(part 1 of 2)
# Autodesk Inventor assembly: printer
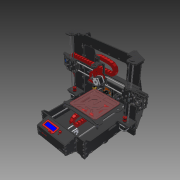
[picture p0: Inventor's stored thumbnail of the model, 180x180]
Saved by Autodesk Inventor 2014 (Build 180170000, 170)
## iProperties
Created: 2014-01-09
Part Number: printer
Document SubType Name: Assembly
Designer: buben
Author: buben
## Documents named in this file (53)
- C:\Users\buben\Documents\GitHub\bacon\inventor files\assemblies\printer.iam
- C:\Users\buben\Documents\GitHub\bacon\inventor files\printer parts\brace_left.ipt
- C:\Users\buben\Documents\GitHub\bacon\inventor files\printer parts\bottom.ipt
- C:\Users\buben\Documents\GitHub\bacon\inventor files\printer parts\brace_right.ipt
- C:\Users\buben\Documents\GitHub\bacon\inventor files\printer parts\front.ipt
- C:\Users\buben\Documents\GitHub\bacon\inventor files\printer parts\back.ipt
- C:\Users\buben\Documents\GitHub\bacon\inventor files\printer parts\frame.ipt
- C:\Users\buben\Documents\GitHub\bacon\inventor files\printer parts\z_motor_brace.ipt
- C:\Users\buben\Documents\GitHub\bacon\inventor files\printer parts\z_motor_mount.ipt
- C:\Users\buben\Documents\GitHub\bacon\inventor files\printer parts\y_axis_cap.ipt
- C:\Users\buben\Documents\GitHub\bacon\inventor files\printer parts\z_rod_stopper_bottom.ipt
- C:\Users\buben\Documents\GitHub\bacon\inventor files\3rd party components\nema_17_stepper\Imported Components\NEMA 17\NEMA 17.iam
- C:\Users\buben\Documents\GitHub\bacon\inventor files\utils\z_axis_rod.ipt
- C:\Users\buben\Documents\GitHub\bacon\inventor files\utils\z_threaded_rod.ipt
- C:\Users\buben\Documents\GitHub\bacon\inventor files\utils\y_axis_rod.ipt
- C:\Users\buben\Documents\GitHub\bacon\inventor files\printer parts\z_axis_top.ipt
- C:\Users\buben\Documents\GitHub\bacon\inventor files\printer parts\z_axis_top_cap.ipt
- C:\Users\buben\Documents\GitHub\bacon\inventor files\printer parts\frame_brace_top.ipt
- C:\Users\buben\Documents\GitHub\bacon\inventor files\utils\washer_m4.ipt
- C:\Users\buben\Documents\Inventor\Content Center Files\R2014\en-US\ISO 4762(2)\ISO 4762 - M4 x 20ISO.ipt
- C:\Users\buben\Documents\Inventor\Content Center Files\R2014\en-US\DIN 985\DIN 985 - M4.ipt
- C:\Users\buben\Documents\Inventor\Content Center Files\R2014\en-US\ISO 7040\ISO 7040 - M4.ipt
- C:\Users\buben\Documents\GitHub\bacon\inventor files\printer parts\wiring_brace.ipt
- C:\Users\buben\Documents\GitHub\bacon\inventor files\utils\washer_m3.ipt
- C:\Users\buben\Documents\Inventor\Content Center Files\R2014\en-US\ISO 4762(2)\ISO 4762 - M3 x 16ISO.ipt
- C:\Users\buben\Documents\GitHub\bacon\inventor files\3rd party components\PC Fan\Imported Components\PC Fan\PC Fan.iam
- C:\Users\buben\Documents\GitHub\bacon\inventor files\3rd party components\fan guard\Imported Components\User Library-Fan Guard\User Library-Fan Guard.ipt
- C:\Users\buben\Documents\GitHub\bacon\inventor files\printer parts\y_carriage_belt_iddler.ipt
- C:\Users\buben\Documents\GitHub\bacon\inventor files\printer parts\y_carriage_belt_iddler_holder.ipt
- C:\Users\buben\Documents\GitHub\bacon\inventor files\3rd party components\bearing_608\Imported Components\608RS\608RS.ipt
- C:\Users\buben\Documents\GitHub\bacon\inventor files\utils\belt_guide.ipt
- C:\Users\buben\Documents\GitHub\bacon\inventor files\utils\washer_m8.ipt
- C:\Users\buben\Documents\Inventor\Content Center Files\R2014\en-US\ISO 7040\ISO 7040 - M8.ipt
- C:\Users\buben\Documents\Inventor\Content Center Files\R2014\en-US\ISO 4762(2)\ISO 4762 - M8 x 40ISO.ipt
- C:\Users\buben\Documents\Inventor\Content Center Files\R2014\en-US\ISO 4762(2)\ISO 4762 - M4 x 30ISO.ipt
- C:\Users\buben\Documents\GitHub\bacon\inventor files\printer parts\y_motor_mount.ipt
- C:\Users\buben\Documents\GitHub\bacon\inventor files\printer parts\y_motor_mount_brace.ipt
- C:\Users\buben\Documents\GitHub\bacon\inventor files\printer parts\motor_spacer.ipt
- C:\Users\buben\Documents\GitHub\bacon\inventor files\3rd party components\nema_17_stepper\Imported Components\NEMA 17 with T5 Pulley\NEMA 17 with T5 Pulley.iam
- C:\Users\buben\Documents\GitHub\bacon\inventor files\assemblies\y_carryage.iam
- C:\Users\buben\Documents\GitHub\bacon\inventor files\assemblies\x_axis.iam
- C:\Users\buben\Documents\GitHub\bacon\inventor files\3rd party components\iec_plug_socket\Imported Components\IEC inlet\IEC inlet.ipt
- C:\Users\buben\Documents\GitHub\bacon\inventor files\utils\z_axis_cable_mount_b.ipt
- C:\Users\buben\Documents\GitHub\bacon\inventor files\utils\cable_chain_22.ipt
- C:\Users\buben\Documents\GitHub\bacon\inventor files\utils\z_axis_cable_mount_a.ipt
- C:\Users\buben\Documents\GitHub\bacon\inventor files\utils\y_axis_cable_mount_b.ipt
- C:\Users\buben\Documents\GitHub\bacon\inventor files\utils\x_axis_cable_mount_a.ipt
- C:\Users\buben\Documents\GitHub\bacon\inventor files\utils\z_axis_coupling_silicone_hose.ipt
- C:\Users\buben\Documents\GitHub\bacon\inventor files\printer parts\y_axis_cap_front_panel.ipt
- C:\Users\buben\Documents\GitHub\bacon\inventor files\assemblies\front_panel_2004.iam
- C:\Users\buben\Documents\GitHub\bacon\inventor files\utils\coupling_tie.ipt
- C:\Users\buben\Documents\GitHub\bacon\inventor files\utils\coupling_tie_belt.ipt
- C:\Users\buben\Documents\Inventor\Content Center Files\R2014\en-US\Screw F-Z GOST R ISO 7050-93\Screw ST4.2x16-F-Z GOST R ISO 7050-93.ipt
## Components (484 placed, 52 different names)
1. brace_left:1 — Mate:1, Mate:2, Mate:3, Mate:4, Mate:5, Flush:1, Mate:8, Mate:9, Mate:10, Mate:11, Mate:13, Mate:14, Mate:15, Mate:16, Mate:23, Mate:24, Mate:25, Mate:78, Mate:79, Flush:3, Mate:123, Mate:205, Mate:207, Mate:506, Flush:10
2. bottom:1 — Mate:4, Mate:5, Flush:1, Mate:6, Flush:2, Mate:7, Mate:12, Mate:80, Mate:91, Mate:484, Mate:485, Mate:510
3. brace_right:1 — Mate:6, Flush:2, Mate:7, Mate:26, Mate:28, Mate:70, Mate:90, Mate:184, Mate:202, Mate:204, Mate:211, Mate:212, Mate:341, Mate:342, Mate:360, Mate:500, Mate:501, Mate:502
4. front:1 — Mate:8, Mate:9, Mate:10, Mate:84, Mate:85, Mate:86, Mate:87, Mate:135, Mate:304, Mate:305, Mate:306, Mate:307, Mate:308, Mate:309, Mate:310, Mate:517, Mate:518, Mate:519, Mate:520, Angle:97, Angle:98, Mate:521, Mate:522, Mate:523, Mate:524, Mate:525, Mate:526, Mate:527, Mate:528, Mate:529, Mate:531, Mate:533, Mate:535, Mate:545, Flush:14, Mate:546
5. back:1 — Mate:11, Mate:12, Mate:13, Mate:35, Mate:36, Mate:37, Mate:38, Mate:39, Mate:40, Insert:3, Insert:4, Mate:255, Mate:256, Mate:257, Mate:258, Mate:286, Mate:287, Mate:288, Mate:289, Mate:290, Mate:291, Mate:292, Mate:511, Insert:188, Insert:189, Insert:190, Insert:191
6. frame:1 — Mate:14, Mate:15, Mate:16, Mate:17, Mate:18, Mate:19, Mate:20, Mate:21, Mate:22, Mate:27, Mate:57, Mate:58, Mate:59, Mate:60, Mate:61, Mate:62, Mate:69, Mate:71, Flush:4, Mate:121, Mate:122, Mate:168, Mate:169, Mate:170, Mate:171, Mate:172, Mate:173, Mate:203, Mate:206, Mate:208, Mate:209, Mate:362, Mate:364, Angle:99, Angle:100
7. z_motor_brace:1 — Mate:20, Mate:21, Mate:22
8. z_motor_brace:2 — Mate:17, Mate:18, Mate:19, Mate:174, Mate:176
9. z_motor_mount:1 — Mate:23, Mate:24, Mate:25, Mate:44, Mate:45, Mate:46, Mate:52, Insert:2
10. z_motor_mount:2 — Mate:26, Mate:27, Mate:28, Mate:41, Mate:42, Mate:43, Insert:1, Mate:160, Mate:161, Mate:162, Mate:163, Mate:164, Mate:165, Mate:166, Mate:167, Mate:180, Mate:182, Mate:220, Mate:221, Mate:222, Mate:223, Mate:224, Mate:225, Mate:226, Mate:227
11. y_axis_cap:2 — Mate:35, Mate:39, Mate:40
12. y_axis_cap:3 — Mate:36, Mate:37, Mate:38
13. z_rod_stopper_bottom:1 — Mate:44, Mate:45, Mate:46, Mate:50, Mate:51
14. z_rod_stopper_bottom:2 — Mate:41, Mate:42, Mate:43, Mate:47, Mate:48, Mate:49, Mate:178, Mate:186
15. NEMA 17:1 [sub-assembly] — Mate:47, Mate:48, Mate:49, Mate:53, Mate:54, Mate:514
16. NEMA 17:2 [sub-assembly] — Mate:50, Mate:51, Mate:52, Mate:55, Mate:56
17. z_axis_rod:1 — Insert:1, Mate:340
18. z_axis_rod:2 — Insert:2, Mate:339
19. z_threaded_rod:1 — Mate:55, Mate:56, Mate:515, Mate:516
20. z_threaded_rod:2 — Mate:53, Mate:54, Mate:513
21. y_axis_rod:1 — Insert:3, Mate:338
22. y_axis_rod:2 — Insert:4, Mate:337
23. z_axis_top:1 — Mate:57, Mate:58, Mate:59, Mate:63, Mate:67, Mate:68
24. z_axis_top:2 — Mate:60, Mate:61, Mate:62, Mate:64, Mate:65, Mate:66, Mate:354, Mate:355, Mate:356, Mate:357, Mate:358, Mate:359, Mate:366, Mate:368
25. z_axis_top_cap:1 — Mate:63, Mate:67, Mate:68
26. z_axis_top_cap:2 — Mate:64, Mate:65, Mate:66, Mate:350, Mate:351, Mate:352, Mate:353
27. frame_brace_top:1 — Mate:69, Mate:70, Mate:71, Mate:343
28. DIN 985 - replaced by DIN EN ISO 10511 M4:12
29. CSN 02 1702 B B 4,3:30 — Insert:9
30. CSN 02 1702 B B 4,3:31 — Mate:106, Mate:108
31. ISO 4762 M4 x 20:15 — Mate:106, Insert:9, Mate:107
32. DIN EN ISO 7040 M4:6 — Mate:107, Mate:108
33. DIN EN ISO 7040 M4:7
34. CSN 02 1702 B B 4,3:32
35. ISO 4762 M4 x 20:16
36. CSN 02 1702 B B 4,3:33
37. DIN EN ISO 7040 M4:8
38. CSN 02 1702 B B 4,3:34
39. ISO 4762 M4 x 20:17
40. CSN 02 1702 B B 4,3:35
41. CSN 02 1702 B B 4,3:42 — Insert:10
42. CSN 02 1702 B B 4,3:43 — Insert:11
43. CSN 02 1702 B B 4,3:44 — Mate:109, Mate:112
44. CSN 02 1702 B B 4,3:45 — Mate:110, Mate:114
45. ISO 4762 M4 x 20:21 — Mate:109, Insert:10, Mate:111
46. ISO 4762 M4 x 20:22 — Mate:110, Insert:11, Mate:113
47. DIN EN ISO 7040 M4:12 — Mate:111, Mate:112
48. DIN EN ISO 7040 M4:13 — Mate:113, Mate:114
49. DIN EN ISO 7040 M4:14
50. CSN 02 1702 B B 4,3:46
51. ISO 4762 M4 x 20:23
52. CSN 02 1702 B B 4,3:47
53. DIN EN ISO 7040 M4:15
54. CSN 02 1702 B B 4,3:48
55. ISO 4762 M4 x 20:24
56. CSN 02 1702 B B 4,3:49
57. CSN 02 1702 B B 4,3:50 — Mate:115, Mate:116
58. ISO 4762 M4 x 20:25 — Mate:115, Mate:117
59. DIN EN ISO 7040 M4:16 — Mate:116, Mate:117
60. DIN EN ISO 7040 M4:17
61. CSN 02 1702 B B 4,3:51
62. ISO 4762 M4 x 20:26
63. CSN 02 1702 B B 4,3:52
64. DIN EN ISO 7040 M4:18
65. CSN 02 1702 B B 4,3:53
66. ISO 4762 M4 x 20:27
67. CSN 02 1702 B B 4,3:54
68. ISO 4762 M4 x 20:28
69. CSN 02 1702 B B 4,3:55
70. CSN 02 1702 B B 4,3:56
71. DIN EN ISO 7040 M4:19
72. ISO 4762 M4 x 20:29
73. CSN 02 1702 B B 4,3:57
74. CSN 02 1702 B B 4,3:58
75. DIN EN ISO 7040 M4:20
76. ISO 4762 M4 x 20:30
77. CSN 02 1702 B B 4,3:59
78. CSN 02 1702 B B 4,3:60
79. DIN EN ISO 7040 M4:21
80. ISO 4762 M4 x 20:35 — Mate:118, Insert:12, Mate:119
81. CSN 02 1702 B B 4,3:69 — Mate:118, Mate:120
82. CSN 02 1702 B B 4,3:70 — Insert:12
83. DIN EN ISO 7040 M4:26 — Mate:119, Mate:120
84. ISO 4762 M4 x 20:36
85. CSN 02 1702 B B 4,3:71
86. CSN 02 1702 B B 4,3:72
87. DIN EN ISO 7040 M4:27
88. ISO 4762 M4 x 20:37
89. CSN 02 1702 B B 4,3:73
90. CSN 02 1702 B B 4,3:74
91. DIN EN ISO 7040 M4:28
92. ISO 4762 M4 x 20:38
93. CSN 02 1702 B B 4,3:75
94. CSN 02 1702 B B 4,3:76
95. DIN EN ISO 7040 M4:29
96. ISO 4762 M4 x 20:39
97. CSN 02 1702 B B 4,3:77
98. CSN 02 1702 B B 4,3:78
99. DIN EN ISO 7040 M4:30
100. CSN 02 1702 B B 4,3:89 — Insert:14
101. CSN 02 1702 B B 4,3:90 — Mate:127, Mate:129
102. ISO 4762 M4 x 20:45 — Mate:127, Insert:14, Mate:128
103. DIN EN ISO 7040 M4:36 — Mate:128, Mate:129
104. ISO 4762 M4 x 20:46
105. CSN 02 1702 B B 4,3:91
106. CSN 02 1702 B B 4,3:92
107. DIN EN ISO 7040 M4:37
108. ISO 4762 M4 x 20:47
109. CSN 02 1702 B B 4,3:93
110. CSN 02 1702 B B 4,3:94
111. DIN EN ISO 7040 M4:38
112. ISO 4762 M4 x 20:48
113. CSN 02 1702 B B 4,3:95
114. CSN 02 1702 B B 4,3:96
115. DIN EN ISO 7040 M4:39
116. ISO 4762 M4 x 20:49
117. CSN 02 1702 B B 4,3:97
118. CSN 02 1702 B B 4,3:98
119. DIN EN ISO 7040 M4:40
120. CSN 02 1702 B B 4,3:100 — Insert:15
121. CSN 02 1702 B B 4,3:102 — Mate:135, Mate:137, Mate:138
122. ISO 4762 M4 x 20:51 — Insert:15, Mate:137, Mate:139
123. DIN EN ISO 7040 M4:41 — Mate:138, Mate:139
124. CSN 02 1702 B B 4,3:104 — Insert:18
125. CSN 02 1702 B B 4,3:106 — Mate:143, Mate:145
126. ISO 4762 M4 x 20:53 — Mate:143, Insert:18, Mate:144
127. DIN EN ISO 7040 M4:43 — Mate:144, Mate:145
128. CSN 02 1702 B B 4,3:107 — Insert:19
129. CSN 02 1702 B B 4,3:108 — Insert:20
130. CSN 02 1702 B B 4,3:109 — Mate:148, Mate:153
131. CSN 02 1702 B B 4,3:110 — Mate:149, Mate:151
132. ISO 4762 M4 x 20:54 — Mate:148, Insert:19, Mate:152
133. ISO 4762 M4 x 20:55 — Mate:149, Insert:20, Mate:150
134. DIN EN ISO 7040 M4:45 — Mate:150, Mate:151
135. DIN EN ISO 7040 M4:46 — Mate:152, Mate:153
136. CSN 02 1702 B B 4,3:111 — Insert:21
137. CSN 02 1702 B B 4,3:112 — Insert:22
138. CSN 02 1702 B B 4,3:113 — Mate:154, Mate:158
139. CSN 02 1702 B B 4,3:114 — Mate:155, Mate:156
140. ISO 4762 M4 x 20:56 — Insert:21, Mate:154, Mate:159
141. ISO 4762 M4 x 20:57 — Insert:22, Mate:155, Mate:157
142. DIN EN ISO 7040 M4:47 — Mate:156, Mate:157
143. DIN EN ISO 7040 M4:48 — Mate:158, Mate:159
144. CSN 02 1702 B B 4,3:115 — Mate:176, Mate:177, Mate:190
145. CSN 02 1702 B B 4,3:116 — Mate:164, Mate:165, Insert:25
146. CSN 02 1702 B B 4,3:117 — Mate:172, Mate:173, Insert:29
147. CSN 02 1702 B B 4,3:118 — Mate:182, Mate:183, Mate:196
148. CSN 02 1702 B B 4,3:119 — Mate:178, Mate:179, Mate:188
149. CSN 02 1702 B B 4,3:120 — Mate:162, Mate:163, Insert:23
150. CSN 02 1702 B B 4,3:121 — Mate:160, Mate:161, Insert:24
151. CSN 02 1702 B B 4,3:122 — Mate:166, Mate:167, Insert:26
152. CSN 02 1702 B B 4,3:123 — Mate:168, Mate:169, Insert:27
153. CSN 02 1702 B B 4,3:124 — Mate:170, Mate:171, Insert:28
154. CSN 02 1702 B B 4,3:125 — Mate:174, Mate:175, Mate:192
155. CSN 02 1702 B B 4,3:126 — Mate:184, Mate:185, Mate:198
156. CSN 02 1702 B B 4,3:127 — Mate:186, Mate:187, Mate:200
157. CSN 02 1702 B B 4,3:128 — Mate:180, Mate:181, Mate:194
158. ISO 4762 M4 x 20:58 — Insert:28, Mate:183, Mate:197
159. ISO 4762 M4 x 20:59 — Insert:29, Mate:175, Mate:193
160. ISO 4762 M4 x 20:60 — Insert:27, Mate:181, Mate:195
161. ISO 4762 M4 x 20:61 — Insert:26, Mate:187, Mate:201
162. ISO 4762 M4 x 20:62 — Insert:25, Mate:185, Mate:199
163. ISO 4762 M4 x 20:63 — Insert:24, Mate:179, Mate:189
164. ISO 4762 M4 x 20:64 — Insert:23, Mate:177, Mate:191
165. DIN EN ISO 7040 M4:49 — Mate:200, Mate:201
166. DIN EN ISO 7040 M4:50 — Mate:198, Mate:199
167. DIN EN ISO 7040 M4:51 — Mate:188, Mate:189
168. DIN EN ISO 7040 M4:52 — Mate:192, Mate:193
169. DIN EN ISO 7040 M4:53 — Mate:194, Mate:195
170. DIN EN ISO 7040 M4:54 — Mate:190, Mate:191
171. DIN EN ISO 7040 M4:55 — Mate:196, Mate:197
172. wiring_brace:1 — Mate:202, Mate:203, Mate:204, Mate:210, Mate:213
173. wiring_brace:2 — Mate:205, Mate:206, Mate:207
174. CSN 02 1702 B B 4,3:129 — Mate:211, Mate:212, Insert:31
175. CSN 02 1702 B B 4,3:130 — Mate:213, Mate:215, Mate:218
176. CSN 02 1702 B B 4,3:131 — Mate:210, Mate:214, Mate:216
177. CSN 02 1702 B B 4,3:132 — Mate:208, Mate:209, Insert:30
178. ISO 4762 M4 x 20:65 — Insert:30, Mate:214, Mate:217
179. ISO 4762 M4 x 20:66 — Insert:31, Mate:215, Mate:219
180. DIN EN ISO 7040 M4:56 — Mate:218, Mate:219
181. DIN EN ISO 7040 M4:57 — Mate:216, Mate:217
182. CSN 02 1702 B B 3,2:1 — Mate:222, Mate:227, Insert:35
183. CSN 02 1702 B B 3,2:2 — Mate:221, Mate:224, Insert:33
184. CSN 02 1702 B B 3,2:3 — Mate:220, Mate:226, Insert:34
185. CSN 02 1702 B B 3,2:4 — Mate:223, Mate:225, Insert:32
186. ISO 4762 M3 x 16:1 — Insert:33
187. ISO 4762 M3 x 16:2 — Insert:32
188. ISO 4762 M3 x 16:3 — Insert:34
189. ISO 4762 M3 x 16:4 — Insert:35
190. CSN 02 1702 B B 4,3:133 — Mate:234, Mate:246
191. CSN 02 1702 B B 4,3:134 — Insert:40
192. CSN 02 1702 B B 4,3:135 — Insert:37
193. CSN 02 1702 B B 4,3:136 — Mate:228, Mate:248
194. CSN 02 1702 B B 4,3:137 — Mate:233, Mate:240
195. CSN 02 1702 B B 4,3:138 — Insert:42
196. CSN 02 1702 B B 4,3:139 — Insert:41
197. CSN 02 1702 B B 4,3:140 — Insert:39
198. CSN 02 1702 B B 4,3:141 — Insert:38
199. CSN 02 1702 B B 4,3:142 — Insert:36
200. CSN 02 1702 B B 4,3:143 — Mate:229, Mate:242
201. CSN 02 1702 B B 4,3:144 — Mate:232, Mate:238
202. CSN 02 1702 B B 4,3:145 — Mate:231, Mate:236
203. CSN 02 1702 B B 4,3:146 — Mate:230, Mate:244
204. ISO 4762 M4 x 20:67 — Mate:228, Insert:36, Mate:247
205. ISO 4762 M4 x 20:68 — Mate:229, Insert:37, Mate:241
206. ISO 4762 M4 x 20:69 — Mate:230, Insert:38, Mate:243
207. ISO 4762 M4 x 20:70 — Mate:231, Insert:39, Mate:235
208. ISO 4762 M4 x 20:71 — Mate:232, Insert:40, Mate:237
209. ISO 4762 M4 x 20:72 — Mate:233, Insert:41, Mate:239
210. ISO 4762 M4 x 20:73 — Mate:234, Insert:42, Mate:245
211. DIN EN ISO 7040 M4:58 — Mate:235, Mate:236
212. DIN EN ISO 7040 M4:59 — Mate:237, Mate:238
213. DIN EN ISO 7040 M4:60 — Mate:239, Mate:240
214. DIN EN ISO 7040 M4:61 — Mate:241, Mate:242
215. DIN EN ISO 7040 M4:62 — Mate:243, Mate:244
216. DIN EN ISO 7040 M4:63 — Mate:245, Mate:246
217. DIN EN ISO 7040 M4:64 — Mate:247, Mate:248
218. CSN 02 1702 B B 4,3:147 — Insert:44
219. CSN 02 1702 B B 4,3:148 — Mate:250, Mate:252
220. CSN 02 1702 B B 4,3:149 — Mate:249, Mate:254
221. CSN 02 1702 B B 4,3:150 — Insert:43
222. ISO 4762 M4 x 20:74 — Mate:249, Insert:43, Mate:253
223. ISO 4762 M4 x 20:75 — Mate:250, Insert:44, Mate:251
224. DIN EN ISO 7040 M4:65 — Mate:251, Mate:252
225. DIN EN ISO 7040 M4:66 — Mate:253, Mate:254
226. CSN 02 1702 B B 3,2:5 — Insert:48
227. CSN 02 1702 B B 3,2:6 — Insert:45
228. CSN 02 1702 B B 3,2:7 — Insert:47
229. CSN 02 1702 B B 3,2:8 — Insert:46
230. ISO 4762 M3 x 16:5 — Insert:45
231. ISO 4762 M3 x 16:6 — Insert:46
232. ISO 4762 M3 x 16:7 — Insert:47
233. ISO 4762 M3 x 16:8 — Insert:48
234. PC Fan:1 [sub-assembly] — Mate:255, Mate:256, Mate:257
235. User Library-Fan Guard:1 — Mate:258
236. y_carriage_belt_iddler:1 — Mate:262, Mate:263, Mate:264, Mate:278, Mate:282, Mate:283, Mate:288
237. y_carriage_belt_iddler:2 — Mate:259, Mate:260, Mate:261, Mate:279, Mate:280, Mate:281, Mate:286, Mate:287
238. y_carriage_belt_iddler_holder:1 — Mate:259, Mate:260, Mate:261, Mate:262, Mate:263, Mate:264, Mate:293, Mate:294
239. 608RS:1 — Mate:265, Mate:266, Mate:269, Mate:274, Mate:275, Mate:276, Mate:277, Mate:279
240. belt_guide:1 — Mate:265, Mate:266, Mate:267, Mate:268
241. belt_guide:2 — Mate:267, Mate:268, Mate:269
242. CSN 02 1702 B B 8,4:1 — Mate:280, Mate:281, Mate:284
243. CSN 02 1702 B B 8,4:2 — Mate:282, Mate:283, Insert:49
244. CSN 02 1702 B B 8,4:3 — Mate:272, Mate:273
245. CSN 02 1702 B B 8,4:4 — Mate:272, Mate:273, Mate:274, Mate:275
246. CSN 02 1702 B B 8,4:5 — Mate:270, Mate:271, Mate:276, Mate:277
247. CSN 02 1702 B B 8,4:6 — Mate:270, Mate:271, Mate:278
248. ISO 4762 M8 x 40:1 — Insert:49, Mate:285
249. DIN EN ISO 7040 M8:1 — Mate:284, Mate:285
250. CSN 02 1702 B B 4,3:151 — Mate:294, Mate:295, Mate:297
251. CSN 02 1702 B B 4,3:152 — Mate:289, Mate:292, Insert:50
252. CSN 02 1702 B B 4,3:153 — Mate:290, Mate:291, Insert:51
253. CSN 02 1702 B B 4,3:154 — Mate:293, Mate:296, Mate:299
254. ISO 4762 M4 x 30:1 — Insert:50, Mate:296, Mate:300
255. ISO 4762 M4 x 30:2 — Insert:51, Mate:295, Mate:298
256. DIN EN ISO 7040 M4:67 — Mate:299, Mate:300
257. DIN EN ISO 7040 M4:68 — Mate:297, Mate:298
258. y_motor_mount:1 — Mate:301, Mate:302, Mate:303, Mate:304, Mate:306, Mate:311, Mate:312, Mate:317, Mate:328, Tangent:1, Tangent:2, Mate:329, Mate:330, Mate:331, Mate:332, Mate:486
259. y_motor_mount_brace:1 — Mate:301, Mate:302, Mate:303, Mate:305, Mate:313, Mate:315
260. CSN 02 1702 B B 4,3:155 — Mate:315, Mate:316, Mate:323
261. CSN 02 1702 B B 4,3:156 — Mate:317, Mate:318, Mate:319
262. CSN 02 1702 B B 4,3:157 — Mate:311, Mate:312, Insert:54
263. CSN 02 1702 B B 4,3:158 — Mate:313, Mate:314, Mate:321
264. CSN 02 1702 B B 4,3:159 — Mate:307, Mate:310, Insert:53
265. CSN 02 1702 B B 4,3:160 — Mate:308, Mate:309, Insert:52
266. ISO 4762 M4 x 20:76 — Insert:54, Mate:316, Mate:324
267. ISO 4762 M4 x 20:77 — Insert:53, Mate:318, Mate:320
268. ISO 4762 M4 x 20:78 — Insert:52, Mate:314, Mate:322
269. DIN EN ISO 7040 M4:69 — Mate:321, Mate:322
270. DIN EN ISO 7040 M4:70 — Mate:319, Mate:320
271. DIN EN ISO 7040 M4:71 — Mate:323, Mate:324
272. motor_spacer:1 — Mate:325, Mate:326, Mate:327, Mate:328, Tangent:1, Tangent:2, Mate:333, Mate:334, Mate:335, Mate:336
273. NEMA 17 with T5 Pulley:1 [sub-assembly] — Mate:325, Mate:326, Mate:327
274. CSN 02 1702 B B 3,2:9 — Mate:331, Insert:57
275. CSN 02 1702 B B 3,2:10 — Mate:332, Insert:58
276. CSN 02 1702 B B 3,2:11 — Mate:330, Insert:56
277. CSN 02 1702 B B 3,2:12 — Mate:329, Insert:55
278. ISO 4762 M3 x 16:9 — Insert:58, Mate:335
279. ISO 4762 M3 x 16:10 — Insert:57, Mate:336
280. ISO 4762 M3 x 16:11 — Insert:56, Mate:334
281. ISO 4762 M3 x 16:12 — Insert:55, Mate:333
282. y_carryage:1 [sub-assembly] — Mate:337, Mate:338, Mate:507, Flush:12, Flush:13
283. x_axis:1 [sub-assembly] — Mate:339, Mate:340, Mate:503, Mate:504, Mate:505
284. CSN 02 1702 B B 4,3:161 — Mate:341, Mate:342, Insert:59
285. CSN 02 1702 B B 4,3:162 — Mate:343, Mate:344, Mate:345
286. ISO 4762 M4 x 20:79 — Insert:59, Mate:344, Mate:346
287. DIN EN ISO 7040 M4:72 — Mate:345, Mate:346
288. CSN 02 1702 B B 4,3:163 — Insert:60
289. CSN 02 1702 B B 4,3:164 — Mate:347, Mate:349
290. ISO 4762 M4 x 20:80 — Mate:347, Insert:60, Mate:348
291. DIN EN ISO 7040 M4:73 — Mate:348, Mate:349
292. CSN 02 1702 B B 4,3:165 — Mate:362, Mate:363, Mate:373
293. CSN 02 1702 B B 4,3:166 — Mate:364, Mate:365, Mate:371
294. CSN 02 1702 B B 4,3:167 — Mate:366, Mate:367, Mate:375
295. CSN 02 1702 B B 4,3:168 — Mate:368, Mate:377, Mate:378
296. CSN 02 1702 B B 4,3:169 — Mate:360, Mate:361, Mate:369
297. CSN 02 1702 B B 4,3:170 — Mate:356, Mate:357, Insert:61
298. CSN 02 1702 B B 4,3:171 — Mate:355, Mate:359, Insert:62
299. CSN 02 1702 B B 4,3:172 — Mate:350, Mate:353, Insert:65
300. CSN 02 1702 B B 4,3:173 — Mate:354, Mate:358, Insert:63
301. CSN 02 1702 B B 4,3:174 — Mate:351, Mate:352, Insert:64
302. ISO 4762 M4 x 20:81 — Insert:61, Mate:361, Mate:370
303. ISO 4762 M4 x 20:82 — Insert:62, Mate:365, Mate:372
304. ISO 4762 M4 x 20:83 — Insert:63, Mate:363, Mate:374
305. ISO 4762 M4 x 20:84 — Insert:64, Mate:367, Mate:376
306. ISO 4762 M4 x 20:85 — Insert:65, Mate:378, Mate:379
307. DIN EN ISO 7040 M4:74 — Mate:377, Mate:379
308. DIN EN ISO 7040 M4:75 — Mate:375, Mate:376
309. DIN EN ISO 7040 M4:76 — Mate:373, Mate:374
310. DIN EN ISO 7040 M4:77 — Mate:371, Mate:372
311. DIN EN ISO 7040 M4:78 — Mate:369, Mate:370
312. CSN 02 1702 B B 4,3:175 — Mate:382, Mate:390
313. CSN 02 1702 B B 4,3:176 — Mate:381, Mate:392
314. CSN 02 1702 B B 4,3:177 — Mate:383, Mate:388
315. CSN 02 1702 B B 4,3:178 — Mate:384, Mate:386
316. CSN 02 1702 B B 4,3:179 — Mate:380, Mate:394
317. CSN 02 1702 B B 4,3:180 — Insert:66
318. CSN 02 1702 B B 4,3:181 — Insert:67
319. CSN 02 1702 B B 4,3:182 — Insert:70
320. CSN 02 1702 B B 4,3:183 — Insert:68
321. CSN 02 1702 B B 4,3:184 — Insert:69
322. ISO 4762 M4 x 20:86 — Mate:380, Insert:66, Mate:393
323. ISO 4762 M4 x 20:87 — Mate:381, Insert:67, Mate:391
324. ISO 4762 M4 x 20:88 — Mate:382, Insert:68, Mate:389
325. ISO 4762 M4 x 20:89 — Mate:383, Insert:69, Mate:387
326. ISO 4762 M4 x 20:90 — Mate:384, Insert:70, Mate:385
327. DIN EN ISO 7040 M4:79 — Mate:385, Mate:386
328. DIN EN ISO 7040 M4:80 — Mate:387, Mate:388
329. DIN EN ISO 7040 M4:81 — Mate:389, Mate:390
330. DIN EN ISO 7040 M4:82 — Mate:391, Mate:392
331. DIN EN ISO 7040 M4:83 — Mate:393, Mate:394
332. CSN 02 1702 B B 4,3:213 — Mate:484, Mate:485, Insert:85
333. CSN 02 1702 B B 4,3:214 — Mate:486, Mate:487, Mate:488
334. ISO 4762 M4 x 20:105 — Insert:85, Mate:487, Mate:489
335. DIN EN ISO 7040 M4:98 — Mate:488, Mate:489
336. IEC inlet:1 — Mate:500, Mate:501, Mate:502, Insert:192, Insert:193
337. z_axis_cable_mount_b:1 — Mate:503, Mate:504, Mate:505, Insert:133, Angle:48
338. cable_chain_22:28 — Insert:134, Flush:9
339. cable_chain_22:29
340. cable_chain_22:30
341. cable_chain_22:31
342. cable_chain_22:32
343. cable_chain_22:33
344. cable_chain_22:34
345. cable_chain_22:35
346. cable_chain_22:36
347. cable_chain_22:37
348. cable_chain_22:38
349. cable_chain_22:39
350. cable_chain_22:40
351. cable_chain_22:41
352. cable_chain_22:42
353. cable_chain_22:43
354. cable_chain_22:44
355. cable_chain_22:45
356. cable_chain_22:46
357. cable_chain_22:47
358. cable_chain_22:48 — Insert:133, Angle:48
359. z_axis_cable_mount_a:1 — Insert:134, Flush:9, Mate:506, Flush:10
360. y_axis_cable_mount_b:1 — Mate:507, Insert:182, Angle:96, Flush:12, Flush:13
361. cable_chain_22:77 — Insert:183, Flush:11
362. cable_chain_22:78
363. cable_chain_22:79
364. cable_chain_22:80
365. cable_chain_22:81
366. cable_chain_22:82
367. cable_chain_22:83
368. cable_chain_22:84
369. cable_chain_22:85
370. cable_chain_22:86
371. cable_chain_22:87
372. cable_chain_22:88
373. cable_chain_22:89
374. cable_chain_22:90
375. cable_chain_22:91
376. cable_chain_22:92
377. cable_chain_22:93
378. cable_chain_22:94
379. cable_chain_22:95
380. cable_chain_22:96 — Insert:182, Angle:96
381. x_axis_cable_mount_a:1 — Insert:183, Flush:11, Mate:510, Mate:511
382. z_axis_coupling_silicone_hose:1 — Mate:515, Mate:516, Mate:549, Flush:18, Flush:19, Mate:550
383. z_axis_coupling_silicone_hose:2 — Mate:513, Mate:514, Mate:547, Flush:15, Flush:16, Mate:548
384. y_axis_cap_front_panel:1 — Mate:517, Mate:518, Angle:97
385. y_axis_cap_front_panel:2 — Mate:519, Mate:520, Angle:98
386. CSN 02 1702 B B 4,3:215 — Mate:529, Mate:530, Mate:537
387. CSN 02 1702 B B 4,3:216 — Mate:525, Mate:526, Insert:186
388. CSN 02 1702 B B 4,3:217 — Mate:527, Mate:528, Insert:187
389. CSN 02 1702 B B 4,3:218 — Mate:523, Mate:524, Insert:185
390. CSN 02 1702 B B 4,3:219 — Mate:531, Mate:532, Mate:539
391. CSN 02 1702 B B 4,3:220 — Mate:521, Mate:522, Insert:184
392. CSN 02 1702 B B 4,3:221 — Mate:533, Mate:534, Mate:541
393. CSN 02 1702 B B 4,3:222 — Mate:535, Mate:536, Mate:543
394. ISO 4762 M4 x 20:106 — Insert:185, Mate:536, Mate:544
395. ISO 4762 M4 x 20:107 — Insert:186, Mate:530, Mate:538
396. ISO 4762 M4 x 20:108 — Insert:187, Mate:532, Mate:540
397. ISO 4762 M4 x 20:109 — Insert:184, Mate:534, Mate:542
398. DIN EN ISO 7040 M4:99 — Mate:539, Mate:540
399. DIN EN ISO 7040 M4:100 — Mate:537, Mate:538
400. DIN EN ISO 7040 M4:101 — Mate:541, Mate:542
401. DIN EN ISO 7040 M4:102 — Mate:543, Mate:544
402. front_panel_2004:1 [sub-assembly] — Mate:545, Flush:14, Mate:546
403. coupling_tie:1 — Mate:547, Flush:15, Flush:17, Angle:100, Mate:553, Mate:554
404. coupling_tie:2 — Flush:19, Mate:550, Flush:20, Mate:555, Mate:556
405. coupling_tie:3 — Flush:16, Flush:17, Mate:548, Mate:551, Mate:552
406. coupling_tie:4 — Mate:549, Flush:18, Flush:20, Angle:99, Mate:557, Mate:558
407. coupling_tie_belt:1 — Mate:551, Mate:552
408. coupling_tie_belt:2 — Mate:553, Mate:554
409. coupling_tie_belt:3 — Mate:555, Mate:556
410. coupling_tie_belt:4 — Mate:557, Mate:558
411. Screw F-Z GOST R ISO 7050-93 ST4.2x16-F-Z:1 — Insert:192
412. Screw F-Z GOST R ISO 7050-93 ST4.2x16-F-Z:2 — Insert:193
413. Screw F-Z GOST R ISO 7050-93 ST4.2x16-F-Z:3 — Insert:191
414. Screw F-Z GOST R ISO 7050-93 ST4.2x16-F-Z:4 — Insert:190
415. Screw F-Z GOST R ISO 7050-93 ST4.2x16-F-Z:5 — Insert:189
416. Screw F-Z GOST R ISO 7050-93 ST4.2x16-F-Z:6 — Insert:188
417. DIN EN ISO 7040 M4:2 — Mate:102, Mate:103
418. CSN 02 1702 B B 4,3:23 — Mate:90, Mate:94, Mate:102
419. ISO 4762 M4 x 20:11 — Insert:7, Mate:94, Mate:103
420. CSN 02 1702 B B 4,3:21 — Mate:84, Mate:85, Insert:7
421. DIN EN ISO 7040 M4:4
422. CSN 02 1702 B B 4,3:26
423. ISO 4762 M4 x 20:13
424. CSN 02 1702 B B 4,3:27
425. DIN EN ISO 7040 M4:5
426. CSN 02 1702 B B 4,3:28
427. ISO 4762 M4 x 20:14
428. CSN 02 1702 B B 4,3:29
429. ISO 4762 M4 x 20:12 — Insert:8, Mate:95, Mate:105
430. CSN 02 1702 B B 4,3:22 — Mate:86, Mate:87, Insert:8
431. CSN 02 1702 B B 4,3:25 — Mate:91, Mate:95, Mate:104
432. DIN EN ISO 7040 M4:3 — Mate:104, Mate:105
433. ISO 4762 M4 x 20:18
434. CSN 02 1702 B B 4,3:36
435. CSN 02 1702 B B 4,3:37
436. DIN EN ISO 7040 M4:9
437. ISO 4762 M4 x 20:19
438. CSN 02 1702 B B 4,3:38
439. CSN 02 1702 B B 4,3:39
440. DIN EN ISO 7040 M4:10
441. ISO 4762 M4 x 20:20
442. CSN 02 1702 B B 4,3:40
443. CSN 02 1702 B B 4,3:41
444. DIN EN ISO 7040 M4:11
445. ISO 4762 M4 x 20:6 — Insert:6, Mate:81, Mate:101
446. CSN 02 1702 B B 4,3:12 — Mate:78, Mate:79, Insert:6
447. CSN 02 1702 B B 4,3:11 — Mate:80, Mate:81, Mate:100
448. DIN EN ISO 7040 M4:1 — Mate:100, Mate:101
449. ISO 4762 M4 x 20:31
450. CSN 02 1702 B B 4,3:61
451. CSN 02 1702 B B 4,3:62
452. DIN EN ISO 7040 M4:22
453. ISO 4762 M4 x 20:32
454. CSN 02 1702 B B 4,3:63
455. CSN 02 1702 B B 4,3:64
456. DIN EN ISO 7040 M4:23
457. ISO 4762 M4 x 20:33
458. CSN 02 1702 B B 4,3:65
459. CSN 02 1702 B B 4,3:66
460. DIN EN ISO 7040 M4:24
461. ISO 4762 M4 x 20:34
462. CSN 02 1702 B B 4,3:67
463. CSN 02 1702 B B 4,3:68
464. DIN EN ISO 7040 M4:25
465. ISO 4762 M4 x 20:40 — Insert:13, Mate:124, Mate:126
466. CSN 02 1702 B B 4,3:79 — Mate:121, Mate:122, Insert:13
467. CSN 02 1702 B B 4,3:80 — Mate:123, Mate:124, Mate:125
468. DIN EN ISO 7040 M4:31 — Mate:125, Mate:126
469. ISO 4762 M4 x 20:41
470. CSN 02 1702 B B 4,3:81
471. CSN 02 1702 B B 4,3:82
472. DIN EN ISO 7040 M4:32
473. ISO 4762 M4 x 20:42
474. CSN 02 1702 B B 4,3:83
475. CSN 02 1702 B B 4,3:84
476. DIN EN ISO 7040 M4:33
477. ISO 4762 M4 x 20:43
478. CSN 02 1702 B B 4,3:85
479. CSN 02 1702 B B 4,3:86
480. DIN EN ISO 7040 M4:34
481. ISO 4762 M4 x 20:44
482. CSN 02 1702 B B 4,3:87
483. CSN 02 1702 B B 4,3:88
484. DIN EN ISO 7040 M4:35
## Component patterns: (3 elements, first: DIN EN ISO 7040 M4:2 + CSN 02 1702 B B 4,3:23 + ISO 4762 M4 x 20:11 + CSN 02 1702 B B 4,3:21), (4 elements, first: ISO 4762 M4 x 20:12 + CSN 02 1702 B B 4,3:22 + CSN 02 1702 B B 4,3:25 + DIN EN ISO 7040 M4:3), (5 elements, first: ISO 4762 M4 x 20:6 + CSN 02 1702 B B 4,3:12 + CSN 02 1702 B B 4,3:11 + DIN EN ISO 7040 M4:1), (5 elements, first: ISO 4762 M4 x 20:40 + CSN 02 1702 B B 4,3:79 + CSN 02 1702 B B 4,3:80 + DIN EN ISO 7040 M4:31)
## Relationships (607: Mate 423, Insert 121, Angle 45, Flush 16, Tangent 2)
- Mate:1: brace_left:1
- Mate:2: brace_left:1
- Mate:3: brace_left:1
- Mate:4: brace_left:1 ↔ bottom:1
- Mate:5: brace_left:1 ↔ bottom:1
- Flush:1: brace_left:1 ↔ bottom:1
- Mate:6: bottom:1 ↔ brace_right:1
- Flush:2: bottom:1 ↔ brace_right:1
- Mate:7: bottom:1 ↔ brace_right:1
- Mate:8: brace_left:1 ↔ front:1
- Mate:9: brace_left:1 ↔ front:1
- Mate:10: brace_left:1 ↔ front:1
- Mate:11: brace_left:1 ↔ back:1
- Mate:12: bottom:1 ↔ back:1
- Mate:13: brace_left:1 ↔ back:1
- Mate:14: brace_left:1 ↔ frame:1
- Mate:15: brace_left:1 ↔ frame:1
- Mate:16: brace_left:1 ↔ frame:1
- Mate:17: frame:1 ↔ z_motor_brace:2
- Mate:18: frame:1 ↔ z_motor_brace:2
- Mate:19: frame:1 ↔ z_motor_brace:2
- Mate:20: frame:1 ↔ z_motor_brace:1
- Mate:21: frame:1 ↔ z_motor_brace:1
- Mate:22: frame:1 ↔ z_motor_brace:1
- Mate:23: brace_left:1 ↔ z_motor_mount:1
- Mate:24: brace_left:1 ↔ z_motor_mount:1
- Mate:25: brace_left:1 ↔ z_motor_mount:1
- Mate:26: brace_right:1 ↔ z_motor_mount:2
- Mate:27: frame:1 ↔ z_motor_mount:2
- Mate:28: brace_right:1 ↔ z_motor_mount:2
- Mate:35: back:1 ↔ y_axis_cap:2
- Mate:36: back:1 ↔ y_axis_cap:3
- Mate:37: back:1 ↔ y_axis_cap:3
- Mate:38: back:1 ↔ y_axis_cap:3
- Mate:39: back:1 ↔ y_axis_cap:2
- Mate:40: back:1 ↔ y_axis_cap:2
- Mate:41: z_motor_mount:2 ↔ z_rod_stopper_bottom:2
- Mate:42: z_motor_mount:2 ↔ z_rod_stopper_bottom:2
- Mate:43: z_motor_mount:2 ↔ z_rod_stopper_bottom:2
- Mate:44: z_motor_mount:1 ↔ z_rod_stopper_bottom:1
- Mate:45: z_motor_mount:1 ↔ z_rod_stopper_bottom:1
- Mate:46: z_motor_mount:1 ↔ z_rod_stopper_bottom:1
- Mate:47: z_rod_stopper_bottom:2 ↔ NEMA 17:1
- Mate:48: z_rod_stopper_bottom:2 ↔ NEMA 17:1
- Mate:49: z_rod_stopper_bottom:2 ↔ NEMA 17:1
- Mate:50: z_rod_stopper_bottom:1 ↔ NEMA 17:2
- Mate:51: z_rod_stopper_bottom:1 ↔ NEMA 17:2
- Mate:52: z_motor_mount:1 ↔ NEMA 17:2
- Insert:1: z_motor_mount:2 ↔ z_axis_rod:1
- Insert:2: z_motor_mount:1 ↔ z_axis_rod:2
- Mate:53: NEMA 17:1 ↔ z_threaded_rod:2
- Mate:54: NEMA 17:1 ↔ z_threaded_rod:2
- Mate:55: NEMA 17:2 ↔ z_threaded_rod:1
- Mate:56: NEMA 17:2 ↔ z_threaded_rod:1
- Insert:3: back:1 ↔ y_axis_rod:1
- Insert:4: back:1 ↔ y_axis_rod:2
- Mate:57: frame:1 ↔ z_axis_top:1
- Mate:58: frame:1 ↔ z_axis_top:1
- Mate:59: frame:1 ↔ z_axis_top:1
- Mate:60: frame:1 ↔ z_axis_top:2
- Mate:61: frame:1 ↔ z_axis_top:2
- Mate:62: frame:1 ↔ z_axis_top:2
- Mate:63: z_axis_top:1 ↔ z_axis_top_cap:1
- Mate:64: z_axis_top:2 ↔ z_axis_top_cap:2
- Mate:65: z_axis_top:2 ↔ z_axis_top_cap:2
- Mate:66: z_axis_top:2 ↔ z_axis_top_cap:2
- Mate:67: z_axis_top:1 ↔ z_axis_top_cap:1
- Mate:68: z_axis_top:1 ↔ z_axis_top_cap:1
- Mate:69: frame:1 ↔ frame_brace_top:1
- Mate:70: brace_right:1 ↔ frame_brace_top:1
- Mate:71: frame:1 ↔ frame_brace_top:1
- Mate:78: brace_left:1 ↔ CSN 02 1702 B B 4,3:12
- Mate:79: brace_left:1 ↔ CSN 02 1702 B B 4,3:12
- Mate:80: bottom:1 ↔ CSN 02 1702 B B 4,3:11
- Insert:6: ISO 4762 M4 x 20:6 ↔ CSN 02 1702 B B 4,3:12
- Mate:81: ISO 4762 M4 x 20:6 ↔ CSN 02 1702 B B 4,3:11
- Mate:84: front:1 ↔ CSN 02 1702 B B 4,3:21
- Mate:85: front:1 ↔ CSN 02 1702 B B 4,3:21
- Mate:86: front:1 ↔ CSN 02 1702 B B 4,3:22
- Mate:87: front:1 ↔ CSN 02 1702 B B 4,3:22
- Mate:90: brace_right:1 ↔ CSN 02 1702 B B 4,3:23
- Mate:91: bottom:1 ↔ CSN 02 1702 B B 4,3:25
- Insert:7: ISO 4762 M4 x 20:11 ↔ CSN 02 1702 B B 4,3:21
- Insert:8: ISO 4762 M4 x 20:12 ↔ CSN 02 1702 B B 4,3:22
- Mate:94: CSN 02 1702 B B 4,3:23 ↔ ISO 4762 M4 x 20:11
- Mate:95: ISO 4762 M4 x 20:12 ↔ CSN 02 1702 B B 4,3:25
- Flush:3 (167.5 mm): brace_left:1
- Mate:100: CSN 02 1702 B B 4,3:11 ↔ DIN EN ISO 7040 M4:1
- Mate:101: ISO 4762 M4 x 20:6 ↔ DIN EN ISO 7040 M4:1
- Mate:102: DIN EN ISO 7040 M4:2 ↔ CSN 02 1702 B B 4,3:23
- Mate:103: DIN EN ISO 7040 M4:2 ↔ ISO 4762 M4 x 20:11
- Mate:104: CSN 02 1702 B B 4,3:25 ↔ DIN EN ISO 7040 M4:3
- Mate:105: ISO 4762 M4 x 20:12 ↔ DIN EN ISO 7040 M4:3
- Flush:4 (77 mm): frame:1
- Mate:106: CSN 02 1702 B B 4,3:31 ↔ ISO 4762 M4 x 20:15
- Insert:9: CSN 02 1702 B B 4,3:30 ↔ ISO 4762 M4 x 20:15
- Mate:107: ISO 4762 M4 x 20:15 ↔ DIN EN ISO 7040 M4:6
- Mate:108: CSN 02 1702 B B 4,3:31 ↔ DIN EN ISO 7040 M4:6
- Mate:109: CSN 02 1702 B B 4,3:44 ↔ ISO 4762 M4 x 20:21
- Insert:10: CSN 02 1702 B B 4,3:42 ↔ ISO 4762 M4 x 20:21
- Mate:110: CSN 02 1702 B B 4,3:45 ↔ ISO 4762 M4 x 20:22
- Insert:11: CSN 02 1702 B B 4,3:43 ↔ ISO 4762 M4 x 20:22
- Mate:111: ISO 4762 M4 x 20:21 ↔ DIN EN ISO 7040 M4:12
- Mate:112: CSN 02 1702 B B 4,3:44 ↔ DIN EN ISO 7040 M4:12
- Mate:113: ISO 4762 M4 x 20:22 ↔ DIN EN ISO 7040 M4:13
- Mate:114: CSN 02 1702 B B 4,3:45 ↔ DIN EN ISO 7040 M4:13
- Mate:115: CSN 02 1702 B B 4,3:50 ↔ ISO 4762 M4 x 20:25
- Mate:116: CSN 02 1702 B B 4,3:50 ↔ DIN EN ISO 7040 M4:16
- Mate:117: ISO 4762 M4 x 20:25 ↔ DIN EN ISO 7040 M4:16
- Mate:118: ISO 4762 M4 x 20:35 ↔ CSN 02 1702 B B 4,3:69
- Insert:12: ISO 4762 M4 x 20:35 ↔ CSN 02 1702 B B 4,3:70
- Mate:119: ISO 4762 M4 x 20:35 ↔ DIN EN ISO 7040 M4:26
- Mate:120: CSN 02 1702 B B 4,3:69 ↔ DIN EN ISO 7040 M4:26
- Mate:121: frame:1 ↔ CSN 02 1702 B B 4,3:79
- Mate:122: frame:1 ↔ CSN 02 1702 B B 4,3:79
- Insert:13: ISO 4762 M4 x 20:40 ↔ CSN 02 1702 B B 4,3:79
- Mate:123: brace_left:1 ↔ CSN 02 1702 B B 4,3:80
- Mate:124: ISO 4762 M4 x 20:40 ↔ CSN 02 1702 B B 4,3:80
- Mate:125: CSN 02 1702 B B 4,3:80 ↔ DIN EN ISO 7040 M4:31
- Mate:126: ISO 4762 M4 x 20:40 ↔ DIN EN ISO 7040 M4:31
- Mate:127: CSN 02 1702 B B 4,3:90 ↔ ISO 4762 M4 x 20:45
- Insert:14: CSN 02 1702 B B 4,3:89 ↔ ISO 4762 M4 x 20:45
- Mate:128: ISO 4762 M4 x 20:45 ↔ DIN EN ISO 7040 M4:36
- Mate:129: CSN 02 1702 B B 4,3:90 ↔ DIN EN ISO 7040 M4:36
- Mate:135: front:1 ↔ CSN 02 1702 B B 4,3:102
- Insert:15: CSN 02 1702 B B 4,3:100 ↔ ISO 4762 M4 x 20:51
- Mate:137: CSN 02 1702 B B 4,3:102 ↔ ISO 4762 M4 x 20:51
- Mate:138: CSN 02 1702 B B 4,3:102 ↔ DIN EN ISO 7040 M4:41
- Mate:139: ISO 4762 M4 x 20:51 ↔ DIN EN ISO 7040 M4:41
- Mate:143: CSN 02 1702 B B 4,3:106 ↔ ISO 4762 M4 x 20:53
- Insert:18: CSN 02 1702 B B 4,3:104 ↔ ISO 4762 M4 x 20:53
- Mate:144: ISO 4762 M4 x 20:53 ↔ DIN EN ISO 7040 M4:43
- Mate:145: CSN 02 1702 B B 4,3:106 ↔ DIN EN ISO 7040 M4:43
- Mate:148: CSN 02 1702 B B 4,3:109 ↔ ISO 4762 M4 x 20:54
- Insert:19: CSN 02 1702 B B 4,3:107 ↔ ISO 4762 M4 x 20:54
- Mate:149: CSN 02 1702 B B 4,3:110 ↔ ISO 4762 M4 x 20:55
- Insert:20: CSN 02 1702 B B 4,3:108 ↔ ISO 4762 M4 x 20:55
- Mate:150: ISO 4762 M4 x 20:55 ↔ DIN EN ISO 7040 M4:45
- Mate:151: CSN 02 1702 B B 4,3:110 ↔ DIN EN ISO 7040 M4:45
- Mate:152: ISO 4762 M4 x 20:54 ↔ DIN EN ISO 7040 M4:46
- Mate:153: CSN 02 1702 B B 4,3:109 ↔ DIN EN ISO 7040 M4:46
- Insert:21: CSN 02 1702 B B 4,3:111 ↔ ISO 4762 M4 x 20:56
- Mate:154: CSN 02 1702 B B 4,3:113 ↔ ISO 4762 M4 x 20:56
- Insert:22: CSN 02 1702 B B 4,3:112 ↔ ISO 4762 M4 x 20:57
- Mate:155: CSN 02 1702 B B 4,3:114 ↔ ISO 4762 M4 x 20:57
- Mate:156: CSN 02 1702 B B 4,3:114 ↔ DIN EN ISO 7040 M4:47
- Mate:157: ISO 4762 M4 x 20:57 ↔ DIN EN ISO 7040 M4:47
- Mate:158: CSN 02 1702 B B 4,3:113 ↔ DIN EN ISO 7040 M4:48
- Mate:159: ISO 4762 M4 x 20:56 ↔ DIN EN ISO 7040 M4:48
- Mate:160: z_motor_mount:2 ↔ CSN 02 1702 B B 4,3:121
- Mate:161: z_motor_mount:2 ↔ CSN 02 1702 B B 4,3:121
- Mate:162: z_motor_mount:2 ↔ CSN 02 1702 B B 4,3:120
- Mate:163: z_motor_mount:2 ↔ CSN 02 1702 B B 4,3:120
- Mate:164: z_motor_mount:2 ↔ CSN 02 1702 B B 4,3:116
- Mate:165: z_motor_mount:2 ↔ CSN 02 1702 B B 4,3:116
- Mate:166: z_motor_mount:2 ↔ CSN 02 1702 B B 4,3:122
- Mate:167: z_motor_mount:2 ↔ CSN 02 1702 B B 4,3:122
- Mate:168: frame:1 ↔ CSN 02 1702 B B 4,3:123
- Mate:169: frame:1 ↔ CSN 02 1702 B B 4,3:123
- Mate:170: frame:1 ↔ CSN 02 1702 B B 4,3:124
- Mate:171: frame:1 ↔ CSN 02 1702 B B 4,3:124
- Mate:172: frame:1 ↔ CSN 02 1702 B B 4,3:117
- Mate:173: frame:1 ↔ CSN 02 1702 B B 4,3:117
- Insert:23: CSN 02 1702 B B 4,3:120 ↔ ISO 4762 M4 x 20:64
- Insert:24: CSN 02 1702 B B 4,3:121 ↔ ISO 4762 M4 x 20:63
- Insert:25: CSN 02 1702 B B 4,3:116 ↔ ISO 4762 M4 x 20:62
- Insert:26: CSN 02 1702 B B 4,3:122 ↔ ISO 4762 M4 x 20:61
- Insert:27: CSN 02 1702 B B 4,3:123 ↔ ISO 4762 M4 x 20:60
- Insert:28: CSN 02 1702 B B 4,3:124 ↔ ISO 4762 M4 x 20:58
- Insert:29: CSN 02 1702 B B 4,3:117 ↔ ISO 4762 M4 x 20:59
- Mate:174: z_motor_brace:2 ↔ CSN 02 1702 B B 4,3:125
- Mate:175: CSN 02 1702 B B 4,3:125 ↔ ISO 4762 M4 x 20:59
- Mate:176: z_motor_brace:2 ↔ CSN 02 1702 B B 4,3:115